# Autodesk Inventor assembly: Intake Assembly
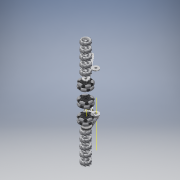
[picture p0: Inventor's stored thumbnail of the model, 180x180]
Saved by Autodesk Inventor 2019.4 (Build 234330000, 330)
## iProperties
Created: 2020-01-28
Part Number: Intake Assembly
Document SubType Name: Assembly
Designer: admin
Mass: 754.204 g
Surface Area: 2733.32 cm^2
Volume: 459.028 cm^3
Density: 1.64305 g/cm^3
Author: admin
## Documents named in this file (8)
- C:\Users\admin\Desktop\FRC 2020 Engineering\GitHub\7738-2020\Robot V2\Intake V2\Intake Assembly.iam
- C:\Users\admin\Desktop\FRC 2020 Engineering\GitHub\7738-2020\Robot V2\Intake V2\Intake Arm.ipt
- C:\Users\admin\Desktop\FRC 2020 Engineering\GitHub\7738-2020\Robot V2\Intake V2\Omni Wheel\3_25_Omni-Directional_Wheel_217-4775.iam
- C:\Users\admin\Desktop\FRC 2020 Engineering\GitHub\7738-2020\Robot V2\Turret\775\775pro_775pro_Connect_and_GT2_Pulley_217-6347 (1).iam
- C:\Users\admin\Desktop\FRC 2020 Engineering\GitHub\7738-2020\Robot V2\Intake V2\Intake Assembly\Design Accelerator\Synchronous Belts Transmission1.iam
- C:\Users\admin\Desktop\FRC 2020 Engineering\GitHub\7738-2020\Robot V2\Intake System\MF148ZZ.ipt
- C:\Users\admin\Desktop\FRC 2020 Engineering\GitHub\7738-2020\Robot V2\Turret\F6800.ipt
- C:\Users\admin\Desktop\FRC 2020 Engineering\GitHub\7738-2020\Robot V2\Intake V2\Mecanum Rad 58x27 Rechts 23 rollen v6.iam
## Components (23 placed, 7 different names)
1. Intake Arm:1 — Mate:1, Mate:2, Mate:3, Mate:4, Mate:5, Mate:6, Mate:7, Mate:9, Mate:10, Mate:11, Mate:12, Mate:13, Mate:14, Mate:15, Mate:18, Mate:23
2. Intake Arm:2 — Mate:1, Mate:2, Mate:3, Mate:8, Mate:16, Mate:17, Mate:19, Mate:20, Mate:21, Mate:22, Mate:42
3. 3_25_Omni-Directional_Wheel_217-4775:1 [sub-assembly] — Mate:4
4. 3_25_Omni-Directional_Wheel_217-4775:2 [sub-assembly] — Mate:5, Mate:28
5. 3_25_Omni-Directional_Wheel_217-4775:3 [sub-assembly] — Mate:6
6. 775pro_775pro_Connect_and_GT2_Pulley_217-6347 (1):1 [sub-assembly] — Mate:9, Mate:10, Mate:23
7. Synchronous Belts Transmission:1 [sub-assembly] — Mate:30
8. MF148ZZ:1 — Mate:12, Mate:14
9. MF148ZZ:2 — Mate:11, Mate:13
10. F6800:1 — Mate:15, Mate:18
11. F6800:2 — Mate:16, Mate:17
12. MF148ZZ:3 — Mate:19, Mate:20, Mate:43
13. MF148ZZ:4 — Mate:21, Mate:22
14. Mecanum Rad 58x27 Rechts 23 rollen v6:4 [sub-assembly] — Mate:24, Mate:25, Mate:29, Mate:31
15. Mecanum Rad 58x27 Rechts 23 rollen v6:5 [sub-assembly] — Mate:24, Mate:33
16. Mecanum Rad 58x27 Rechts 23 rollen v6:6 [sub-assembly] — Mate:25, Mate:26, Mate:27, Mate:31, Mate:32
17. Mecanum Rad 58x27 Rechts 23 rollen v6:7 [sub-assembly] — Mate:26, Mate:28, Mate:32, Mate:33
18. Mecanum Rad 58x27 Rechts 23 rollen v6:8 [sub-assembly] — Mate:27, Mate:29, Mate:30
19. Mecanum Rad 58x27 Rechts 23 rollen v6:9 [sub-assembly]
20. Mecanum Rad 58x27 Rechts 23 rollen v6:10 [sub-assembly]
21. Mecanum Rad 58x27 Rechts 23 rollen v6:11 [sub-assembly]
22. Mecanum Rad 58x27 Rechts 23 rollen v6:12 [sub-assembly]
23. Mecanum Rad 58x27 Rechts 23 rollen v6:13 [sub-assembly] — Mate:42, Mate:43
## Relationships (43: Mate 43)
- Mate:1: Intake Arm:1 ↔ Intake Arm:2
- Mate:2: Intake Arm:1 ↔ Intake Arm:2
- Mate:3 (248.6 mm): Intake Arm:1 ↔ Intake Arm:2
- Mate:4: Intake Arm:1 ↔ 3_25_Omni-Directional_Wheel_217-4775:1
- Mate:5: Intake Arm:1 ↔ 3_25_Omni-Directional_Wheel_217-4775:2
- Mate:6: Intake Arm:1 ↔ 3_25_Omni-Directional_Wheel_217-4775:3
- Mate:7: Intake Arm:1
- Mate:8 (119.3 mm): Intake Arm:2
- Mate:9: Intake Arm:1 ↔ 775pro_775pro_Connect_and_GT2_Pulley_217-6347 (1):1
- Mate:10: Intake Arm:1 ↔ 775pro_775pro_Connect_and_GT2_Pulley_217-6347 (1):1
- Mate:11: Intake Arm:1 ↔ MF148ZZ:2
- Mate:12: Intake Arm:1 ↔ MF148ZZ:1
- Mate:13 (0.2 mm): Intake Arm:1 ↔ MF148ZZ:2
- Mate:14 (0.2 mm): Intake Arm:1 ↔ MF148ZZ:1
- Mate:15: Intake Arm:1 ↔ F6800:1
- Mate:16: Intake Arm:2 ↔ F6800:2
- Mate:17 (0.2 mm): Intake Arm:2 ↔ F6800:2
- Mate:18 (0.2 mm): Intake Arm:1 ↔ F6800:1
- Mate:19: Intake Arm:2 ↔ MF148ZZ:3
- Mate:20 (0.2 mm): Intake Arm:2 ↔ MF148ZZ:3
- Mate:21: Intake Arm:2 ↔ MF148ZZ:4
- Mate:22 (0.2 mm): Intake Arm:2 ↔ MF148ZZ:4
- Mate:23: Intake Arm:1 ↔ 775pro_775pro_Connect_and_GT2_Pulley_217-6347 (1):1
- Mate:24: Mecanum Rad 58x27 Rechts 23 rollen v6:4 ↔ Mecanum Rad 58x27 Rechts 23 rollen v6:5
- Mate:25: Mecanum Rad 58x27 Rechts 23 rollen v6:4 ↔ Mecanum Rad 58x27 Rechts 23 rollen v6:6
- Mate:26: Mecanum Rad 58x27 Rechts 23 rollen v6:6 ↔ Mecanum Rad 58x27 Rechts 23 rollen v6:7
- Mate:27: Mecanum Rad 58x27 Rechts 23 rollen v6:6 ↔ Mecanum Rad 58x27 Rechts 23 rollen v6:8
- Mate:28: 3_25_Omni-Directional_Wheel_217-4775:2 ↔ Mecanum Rad 58x27 Rechts 23 rollen v6:7
- Mate:29 (20 mm): Mecanum Rad 58x27 Rechts 23 rollen v6:4 ↔ Mecanum Rad 58x27 Rechts 23 rollen v6:8
- Mate:30 (5 mm): Synchronous Belts Transmission:1 ↔ Mecanum Rad 58x27 Rechts 23 rollen v6:8
- Mate:31 (20 mm): Mecanum Rad 58x27 Rechts 23 rollen v6:4 ↔ Mecanum Rad 58x27 Rechts 23 rollen v6:6
- Mate:32 (20 mm): Mecanum Rad 58x27 Rechts 23 rollen v6:6 ↔ Mecanum Rad 58x27 Rechts 23 rollen v6:7
- Mate:33 (20 mm): Mecanum Rad 58x27 Rechts 23 rollen v6:5 ↔ Mecanum Rad 58x27 Rechts 23 rollen v6:7
- [Mate]: Mecanum Rad 58x27 Rechts 23 rollen v6:9 ↔ Mecanum Rad 58x27 Rechts 23 rollen v6:10
- [Mate]: Mecanum Rad 58x27 Rechts 23 rollen v6:9 ↔ Mecanum Rad 58x27 Rechts 23 rollen v6:11
- [Mate]: Mecanum Rad 58x27 Rechts 23 rollen v6:11 ↔ Mecanum Rad 58x27 Rechts 23 rollen v6:12
- [Mate]: Mecanum Rad 58x27 Rechts 23 rollen v6:11 ↔ Mecanum Rad 58x27 Rechts 23 rollen v6:13
- [Mate] (20 mm): Mecanum Rad 58x27 Rechts 23 rollen v6:9 ↔ Mecanum Rad 58x27 Rechts 23 rollen v6:13
- [Mate] (20 mm): Mecanum Rad 58x27 Rechts 23 rollen v6:9 ↔ Mecanum Rad 58x27 Rechts 23 rollen v6:11
- [Mate] (20 mm): Mecanum Rad 58x27 Rechts 23 rollen v6:11 ↔ Mecanum Rad 58x27 Rechts 23 rollen v6:12
- [Mate] (20 mm): Mecanum Rad 58x27 Rechts 23 rollen v6:10 ↔ Mecanum Rad 58x27 Rechts 23 rollen v6:12
- Mate:42 (22.5 mm): Intake Arm:2 ↔ Mecanum Rad 58x27 Rechts 23 rollen v6:13
- Mate:43: MF148ZZ:3 ↔ Mecanum Rad 58x27 Rechts 23 rollen v6:13
## Named parameters: d37_d35 = 20 mm, d38_d36 = 20 mm, d39_d32 = 20 mm, d40_d34 = 20 mm, d41_d23 = 0 mm, d42_d24 = 0 mm, d43_d25 = 0 mm, d44_d26 = 0 mm
